# Autodesk Inventor assembly: wheel
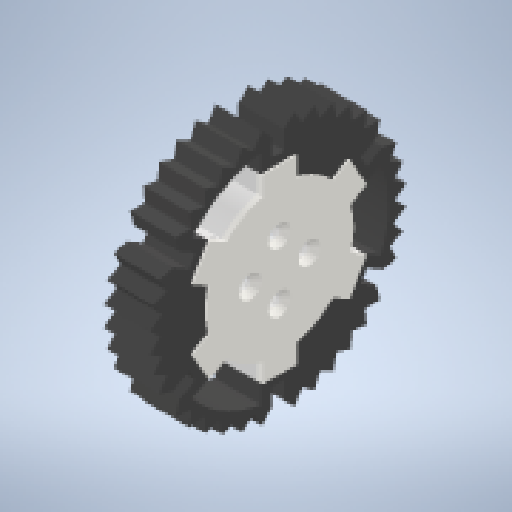
[picture p0: Inventor's stored thumbnail of the model, 512x512]
Saved by Autodesk Inventor 2023 (Build 270158000, 158)
## iProperties
Created: 2026-02-21
Part Number: wheel
Document SubType Name: Assembly
Designer: garin
Author: garin
## Documents named in this file (5)
- C:\Users\garin\OneDrive\Документы\maze\version1\wheel.iam
- C:\Users\garin\OneDrive\Документы\maze\version1\tire.ipt
- C:\Users\garin\OneDrive\Документы\maze\version1\wheel_mold.ipt
- C:\Users\garin\OneDrive\Документы\maze\version1\inside_part_wheel.ipt
- C:\Users\garin\OneDrive\Документы\maze\version1\top_part_wheel.ipt
## Components (4 placed, 4 different names)
1. tire:1 — Заподлицо:1, Заподлицо:2, Заподлицо:3
2. inside_part_wheel:1 — Заподлицо:2, С поворотом:1
3. top_part_wheel:1 — Заподлицо:3, С поворотом:1
4. wheel_mold:1 — Заподлицо:1
## Relationships (4: Flush 3, RevoluteJoint 1)
- Заподлицо:1 [Flush]: tire:1 ↔ wheel_mold:1
- Заподлицо:2 [Flush]: tire:1 ↔ inside_part_wheel:1
- Заподлицо:3 [Flush]: tire:1 ↔ top_part_wheel:1
- С поворотом:1 [RevoluteJoint]: inside_part_wheel:1 ↔ top_part_wheel:1
